# Autodesk Inventor assembly: OpticsTable_Shelf
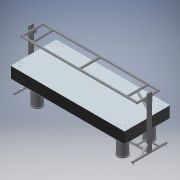
[picture p0: Inventor's stored thumbnail of the model, 180x180]
Saved by Autodesk Inventor 2018 (Build 220112000, 112)
## iProperties
Created: 2018-01-27
Part Number: OpticsTable_Shelf
Document SubType Name: Assembly
Designer: Rich
Author: Rich
## Documents named in this file (23)
- C:\Users\Rich\development\UWaterloo\opticstable_shelf\OpticsTable_Shelf.iam
- C:\Users\Rich\development\UWaterloo\opticstable_shelf\8020-1545-S-1545-S X 54.ipt
- C:\Users\Rich\development\UWaterloo\opticstable_shelf\8020-1515-LS-1515-LS X 24.ipt
- C:\Users\Rich\development\UWaterloo\opticstable_shelf\8020-1515-LS-1515-LS X 21.ipt
- C:\Users\Rich\development\UWaterloo\opticstable_shelf\8020 Original Parts\8020-3660-DEFAULT.ipt
- C:\Users\Rich\development\UWaterloo\opticstable_shelf\8020-1515-LS-1515-LS X 36.ipt
- C:\Users\Rich\development\UWaterloo\opticstable_shelf\8020 Original Parts\8020-2561-$PARTNUMBER.ipt
- C:\Users\Rich\development\UWaterloo\opticstable_shelf\8020 Original Parts\8020-2563-$PARTNUMBER.ipt
- C:\Users\Rich\development\UWaterloo\opticstable_shelf\8020 Original Parts\8020-2190-DEFAULT.ipt
- C:\Users\Rich\development\UWaterloo\opticstable_shelf\8020 Original Parts\8020-2200-DEFAULT.ipt
- C:\Users\Rich\development\UWaterloo\opticstable_shelf\8020 Original Parts\RS2000-410-12.ipt
- C:\Users\Rich\development\UWaterloo\opticstable_shelf\8020 Original Parts\Newport SL 1200-422.ipt
- C:\Users\Rich\development\UWaterloo\opticstable_shelf\8020-1515-LS-1515-LS X 120.ipt
- C:\Users\Rich\development\UWaterloo\opticstable_shelf\8020-1515-LS-1515-LS X 123.ipt
- C:\Users\Rich\development\UWaterloo\opticstable_shelf\8020 Original Parts\8020-3118-DEFAULT.ipt
- C:\Users\Rich\development\UWaterloo\opticstable_shelf\8020 Original Parts\8020-4461-DEFAULT.ipt
- C:\Users\Rich\development\UWaterloo\opticstable_shelf\8020 Original Parts\8020-4336-BLACK-DEFAULT.ipt
- C:\Users\Rich\development\UWaterloo\opticstable_shelf\8020 Original Parts\User Library-ANSI - BHCS - 0.625_5.5.ipt
- C:\Users\Rich\development\UWaterloo\opticstable_shelf\8020 Original Parts\8020-3202-DEFAULT.ipt
- C:\Users\Rich\development\UWaterloo\opticstable_shelf\8020 Original Parts\8020-3065-DEFAULT.ipt
- C:\Users\Rich\development\UWaterloo\opticstable_shelf\8020 Original Parts\8020-2046-DEFAULT.ipt
- C:\Users\Rich\development\UWaterloo\opticstable_shelf\8020 Original Parts\8020-2030-Plain-DEFAULT.ipt
- C:\Users\Rich\development\UWaterloo\opticstable_shelf\8020 Original Parts\8020-3214-DEFAULT.ipt
## Components (107 placed, 22 different names)
1. 8020-1545-S-1545-S X 54:1 — Mate:12, Flush:21, Flush:22, Flush:26, Mate:18, Mate:25, Flush:29, Mate:26, Flush:33, Flush:41, Mate:36, Angle:10, Flush:42, Mate:37, Angle:11, Mate:50, Flush:53, Mate:81, Mate:82, Mate:118, Mate:120, Mate:167, Mate:168, Mate:169
2. 8020-1545-S-1545-S X 54:2 — Mate:2, Flush:4, Flush:18, Flush:20, Flush:21, Mate:15, Mate:16, Mate:21, Flush:27, Mate:23, Flush:34, Flush:39, Mate:34, Angle:8, Flush:40, Mate:35, Angle:9, Mate:49, Flush:52, Mate:79, Mate:80, Mate:125, Mate:126, Mate:170, Mate:171, Mate:172
3. 8020-1515-LS-1515-LS X 24:1 — Flush:61, Mate:60, Flush:62, Mate:61, Flush:63, Flush:64, Mate:129, Mate:179, Flush:93, Flush:94, Mate:180, Flush:95, Flush:96, Tangent:3
4. 8020-1515-LS-1515-LS X 24:2 — Flush:20, Flush:23, Flush:68, Mate:64, Flush:69, Mate:130, Mate:177, Flush:89, Flush:90, Flush:91, Mate:178, Flush:92
5. 8020-1515-LS-1515-LS X 21:1 — Mate:17, Mate:46, Flush:51, Angle:16, Mate:47, Mate:48, Angle:17, Flush:72, Mate:68, Tangent:2, Mate:71
6. 8020-1515-LS-1515-LS X 21:2 — Flush:23, Mate:44, Flush:49, Angle:14, Mate:45, Flush:50, Angle:15, Flush:67, Mate:63
7. 8020-1515-LS-1515-LS X 21:3 — Mate:19, Flush:47, Mate:42, Angle:12, Flush:48, Mate:43, Angle:13, Mate:62, Flush:65, Tangent:1, Mate:67
8. 8020-1515-LS-1515-LS X 36:1 — Mate:12, Flush:19, Flush:22, Mate:24, Mate:27, Flush:30, Mate:38, Flush:43, Mate:39, Flush:44, Flush:77, Mate:75, Mate:175, Flush:85, Flush:86, Mate:176, Flush:87, Flush:88
9. 8020-1515-LS-1515-LS X 36:2 — Mate:1, Mate:2, Flush:4, Flush:18, Flush:19, Mate:20, Mate:22, Flush:28, Mate:40, Flush:45, Mate:41, Flush:46, Mate:72, Flush:75, Mate:173, Flush:81, Flush:82, Mate:174, Flush:83, Flush:84
10. 8020-3660-DEFAULT:1 — Mate:66, Flush:71, Angle:18
11. 8020-3660-DEFAULT:2 — Mate:69, Flush:73, Angle:19
12. 8020-2561-$PARTNUMBER:1 — Mate:22, Mate:23, Flush:28
13. 8020-2561-$PARTNUMBER:2 — Mate:24, Mate:25, Flush:29
14. 8020-2563-$PARTNUMBER:1 — Mate:16, Mate:17, Flush:34, Tangent:1, Mate:67
15. 8020-2563-$PARTNUMBER:2 — Mate:18, Mate:19, Flush:33, Mate:68, Tangent:2
16. 8020-2561-$PARTNUMBER:3 — Mate:26, Mate:27, Flush:30
17. 8020-2561-$PARTNUMBER:4 — Mate:20, Mate:21, Flush:27
18. 8020-2190-DEFAULT:1
19. 8020-2190-DEFAULT:2
20. 8020-2190-DEFAULT:3
21. 8020-3660-DEFAULT:3 — Mate:70, Flush:74, Angle:20
22. 8020-3660-DEFAULT:4 — Mate:65, Flush:70
23. 8020-3660-DEFAULT:9 — Flush:39, Mate:34, Angle:8
24. 8020-3660-DEFAULT:10 — Flush:40, Mate:35, Angle:9
25. 8020-3660-DEFAULT:11 — Flush:41, Mate:36, Angle:10
26. 8020-3660-DEFAULT:12 — Flush:42, Mate:37, Angle:11
27. 8020-2200-DEFAULT:1 — Mate:38, Flush:43
28. 8020-2200-DEFAULT:2 — Mate:39, Flush:44
29. 8020-2200-DEFAULT:3 — Mate:40, Flush:45
30. 8020-2200-DEFAULT:4 — Mate:41, Flush:46
31. 8020-3660-DEFAULT:13 — Flush:47, Mate:42, Angle:12
32. 8020-3660-DEFAULT:14 — Flush:48, Mate:43, Angle:13
33. 8020-3660-DEFAULT:15 — Mate:44, Flush:49, Angle:14
34. 8020-3660-DEFAULT:16 — Mate:45, Flush:50, Angle:15
35. 8020-3660-DEFAULT:17 — Mate:46, Flush:51, Angle:16
36. 8020-3660-DEFAULT:18 — Mate:47, Mate:48, Angle:17
37. 8020-2563-$PARTNUMBER:3 — Mate:49, Flush:52, Flush:76, Mate:73
38. 8020-2563-$PARTNUMBER:4 — Mate:50, Flush:53, Mate:74
39. 8020-2200-DEFAULT:5 — Mate:76, Flush:78
40. 8020-2200-DEFAULT:6 — Flush:79, Mate:77
41. RS2000-410-12:1 — Mate:57, Mate:58, Flush:60
42. 8020-1515-LS-1515-LS X 120:1 — Flush:62, Mate:61, Flush:63, Mate:63, Mate:66, Flush:71, Angle:18, Mate:69, Flush:73, Angle:19, Mate:71
43. 8020-1515-LS-1515-LS X 120:2 — Flush:61, Mate:60, Flush:64, Mate:62, Flush:65, Flush:67, Flush:68, Mate:64, Flush:69, Mate:65, Flush:70, Flush:72, Mate:70, Flush:74, Angle:20
44. 8020-1515-LS-1515-LS X 123:1 — Mate:72, Flush:75, Flush:76, Mate:73, Mate:74, Flush:77, Mate:75, Mate:76, Flush:78, Flush:79, Mate:77, Mate:78, Flush:80
45. 8020-2200-DEFAULT:7 — Mate:78, Flush:80
46. 8020-3118-DEFAULT:1 — Mate:84, Mate:85, Mate:88, Mate:184
47. 8020-4461-DEFAULT:1 — Mate:79, Mate:95, Mate:96, Mate:97, Mate:116, Mate:117, Mate:123, Mate:124, Mate:193, Mate:194
48. 8020-4461-DEFAULT:2 — Mate:80, Mate:83, Mate:88, Mate:89, Mate:127, Mate:128, Mate:195, Mate:196, Mate:198, Mate:200
49. 8020-4461-DEFAULT:3 — Mate:81, Mate:109, Mate:110, Mate:111, Mate:112, Mate:114, Mate:115, Mate:119, Mate:189, Mate:190
50. 8020-4461-DEFAULT:4 — Mate:82, Mate:102, Mate:103, Mate:104, Mate:121, Mate:122, Mate:191, Mate:192, Mate:202, Mate:204
51. 8020-4336-BLACK-DEFAULT:1 — Mate:83, Mate:84, Mate:85, Mate:86, Mate:87, Mate:130, Mate:149, Mate:150, Mate:154, Mate:155, Mate:156
52. 8020-3118-DEFAULT:2 — Mate:86, Mate:87, Mate:89, Mate:185
53. 8020-4336-BLACK-DEFAULT:2 — Mate:91, Mate:92, Mate:93, Mate:94, Mate:95, Mate:151, Mate:152, Mate:153, Mate:157, Mate:158
54. 8020-3118-DEFAULT:3 — Mate:91, Mate:92, Mate:97, Mate:186
55. 8020-3118-DEFAULT:4 — Mate:93, Mate:94, Mate:96, Mate:187
56. 8020-3118-DEFAULT:5 — Mate:98, Mate:99, Mate:104, Mate:181
57. 8020-4336-BLACK-DEFAULT:3 — Mate:98, Mate:99, Mate:100, Mate:101, Mate:102, Mate:129, Mate:159, Mate:160, Mate:161, Mate:162
58. 8020-3118-DEFAULT:6 — Mate:100, Mate:101, Mate:103, Mate:182
59. 8020-4336-BLACK-DEFAULT:4 — Mate:105, Mate:106, Mate:107, Mate:108, Mate:109, Mate:163, Mate:164, Mate:165, Mate:166
60. 8020-3118-DEFAULT:7 — Mate:105, Mate:106, Mate:110, Mate:183
61. 8020-3118-DEFAULT:8 — Mate:107, Mate:108, Mate:111, Mate:188
62. User Library-ANSI - BHCS - 0.625_5.5:1 — Mate:114, Mate:115, Mate:118, Mate:121, Mate:203
63. User Library-ANSI - BHCS - 0.625_5.5:2 — Mate:112, Mate:119, Mate:120, Mate:122, Mate:201
64. User Library-ANSI - BHCS - 0.625_5.5:3 — Mate:117, Mate:124, Mate:125, Mate:128, Mate:199
65. User Library-ANSI - BHCS - 0.625_5.5:4 — Mate:116, Mate:123, Mate:126, Mate:127, Mate:197
66. 8020-3202-DEFAULT:1 — Mate:131, Mate:132
67. 8020-3065-DEFAULT:1 — Mate:131, Mate:132, Mate:159, Mate:160
68. 8020-3202-DEFAULT:2
69. 8020-3065-DEFAULT:2 — Mate:163, Mate:164
70. 8020-3202-DEFAULT:4
71. 8020-3065-DEFAULT:4 — Mate:165, Mate:166
72. 8020-3202-DEFAULT:5
73. 8020-3065-DEFAULT:5 — Mate:161, Mate:162, Tangent:3
74. 8020-3202-DEFAULT:6
75. 8020-3065-DEFAULT:6 — Mate:151, Mate:157, Mate:158
76. 8020-3202-DEFAULT:7
77. 8020-3065-DEFAULT:7 — Mate:150, Mate:155, Mate:156
78. 8020-3202-DEFAULT:8
79. 8020-3065-DEFAULT:8 — Mate:149, Mate:154
80. 8020-3202-DEFAULT:9
81. 8020-3065-DEFAULT:9 — Mate:152, Mate:153
82. 8020-2046-DEFAULT:1 — Mate:167, Mate:168, Mate:169
83. 8020-2046-DEFAULT:2 — Mate:170, Mate:171, Mate:172
84. 8020-2030-Plain-DEFAULT:1 — Mate:180, Flush:95, Flush:96
85. 8020-2030-Plain-DEFAULT:2 — Mate:179, Flush:93, Flush:94
86. 8020-2030-Plain-DEFAULT:3 — Flush:91, Mate:178, Flush:92
87. 8020-2030-Plain-DEFAULT:4 — Mate:177, Flush:89, Flush:90
88. 8020-2030-Plain-DEFAULT:5 — Mate:173, Flush:81, Flush:82
89. 8020-2030-Plain-DEFAULT:6 — Mate:174, Flush:83, Flush:84
90. 8020-2030-Plain-DEFAULT:7 — Mate:175, Flush:85, Flush:86
91. 8020-2030-Plain-DEFAULT:8 — Mate:176, Flush:87, Flush:88
92. 8020-3214-DEFAULT:1 — Mate:181, Mate:191
93. 8020-3214-DEFAULT:2 — Mate:182, Mate:192
94. 8020-3214-DEFAULT:3 — Mate:183, Mate:190
95. 8020-3214-DEFAULT:4 — Mate:185, Mate:196
96. 8020-3214-DEFAULT:5 — Mate:184, Mate:195
97. 8020-3214-DEFAULT:6 — Mate:186, Mate:193
98. 8020-3214-DEFAULT:7 — Mate:187, Mate:194
99. 8020-3214-DEFAULT:8 — Mate:188, Mate:189
100. 8020-3214-DEFAULT:9 — Mate:197, Mate:198
101. 8020-3214-DEFAULT:10 — Mate:199, Mate:200
102. 8020-3214-DEFAULT:11 — Mate:201, Mate:202
103. 8020-3214-DEFAULT:12 — Mate:203, Mate:204
104. Newport SL 1200-422:1 — Mate:57, Mate:58, Flush:60, Mate:59
105. Newport SL 1200-422:2
106. Newport SL 1200-422:3
107. Newport SL 1200-422:4
## Component patterns: (4 elements, first: Newport SL 1200-422:1)
## Relationships (258: Mate 177, Flush 65, Angle 13, Tangent 3)
- Mate:1: 8020-1515-LS-1515-LS X 36:2
- Mate:2: 8020-1545-S-1545-S X 54:2 ↔ 8020-1515-LS-1515-LS X 36:2
- Flush:4: 8020-1545-S-1545-S X 54:2 ↔ 8020-1515-LS-1515-LS X 36:2
- Mate:12: 8020-1545-S-1545-S X 54:1 ↔ 8020-1515-LS-1515-LS X 36:1
- Flush:18 (-400.05 mm): 8020-1545-S-1545-S X 54:2 ↔ 8020-1515-LS-1515-LS X 36:2
- Flush:19: 8020-1515-LS-1515-LS X 36:1 ↔ 8020-1515-LS-1515-LS X 36:2
- Flush:20 (247.65 mm): 8020-1545-S-1545-S X 54:2 ↔ 8020-1515-LS-1515-LS X 24:2
- Flush:21: 8020-1545-S-1545-S X 54:1 ↔ 8020-1545-S-1545-S X 54:2
- Flush:22: 8020-1545-S-1545-S X 54:1 ↔ 8020-1515-LS-1515-LS X 36:1
- Flush:23 (-1530.95 mm): 8020-1515-LS-1515-LS X 24:2 ↔ 8020-1515-LS-1515-LS X 21:2
- Flush:26: 8020-1545-S-1545-S X 54:1
- Mate:15: 8020-1545-S-1545-S X 54:2
- Mate:16: 8020-1545-S-1545-S X 54:2 ↔ 8020-2563-$PARTNUMBER:1
- Mate:17: 8020-1515-LS-1515-LS X 21:1 ↔ 8020-2563-$PARTNUMBER:1
- Mate:18: 8020-1545-S-1545-S X 54:1 ↔ 8020-2563-$PARTNUMBER:2
- Mate:19: 8020-1515-LS-1515-LS X 21:3 ↔ 8020-2563-$PARTNUMBER:2
- Mate:20: 8020-1515-LS-1515-LS X 36:2 ↔ 8020-2561-$PARTNUMBER:4
- Mate:21: 8020-1545-S-1545-S X 54:2 ↔ 8020-2561-$PARTNUMBER:4
- Flush:27: 8020-1545-S-1545-S X 54:2 ↔ 8020-2561-$PARTNUMBER:4
- Mate:22: 8020-1515-LS-1515-LS X 36:2 ↔ 8020-2561-$PARTNUMBER:1
- Mate:23: 8020-1545-S-1545-S X 54:2 ↔ 8020-2561-$PARTNUMBER:1
- Flush:28: 8020-1515-LS-1515-LS X 36:2 ↔ 8020-2561-$PARTNUMBER:1
- Mate:24: 8020-1515-LS-1515-LS X 36:1 ↔ 8020-2561-$PARTNUMBER:2
- Mate:25: 8020-1545-S-1545-S X 54:1 ↔ 8020-2561-$PARTNUMBER:2
- Flush:29: 8020-1545-S-1545-S X 54:1 ↔ 8020-2561-$PARTNUMBER:2
- Mate:26: 8020-1545-S-1545-S X 54:1 ↔ 8020-2561-$PARTNUMBER:3
- Mate:27: 8020-1515-LS-1515-LS X 36:1 ↔ 8020-2561-$PARTNUMBER:3
- Flush:30: 8020-1515-LS-1515-LS X 36:1 ↔ 8020-2561-$PARTNUMBER:3
- Flush:33 (38.1 mm): 8020-1545-S-1545-S X 54:1 ↔ 8020-2563-$PARTNUMBER:2
- Flush:34 (-38.1 mm): 8020-1545-S-1545-S X 54:2 ↔ 8020-2563-$PARTNUMBER:1
- Flush:39: 8020-1545-S-1545-S X 54:2 ↔ 8020-3660-DEFAULT:9
- Mate:34: 8020-1545-S-1545-S X 54:2 ↔ 8020-3660-DEFAULT:9
- Angle:8 (0 deg): 8020-1545-S-1545-S X 54:2 ↔ 8020-3660-DEFAULT:9
- Flush:40: 8020-1545-S-1545-S X 54:2 ↔ 8020-3660-DEFAULT:10
- Mate:35: 8020-1545-S-1545-S X 54:2 ↔ 8020-3660-DEFAULT:10
- Angle:9 (0 deg): 8020-1545-S-1545-S X 54:2 ↔ 8020-3660-DEFAULT:10
- Flush:41: 8020-1545-S-1545-S X 54:1 ↔ 8020-3660-DEFAULT:11
- Mate:36: 8020-1545-S-1545-S X 54:1 ↔ 8020-3660-DEFAULT:11
- Angle:10 (180 deg): 8020-1545-S-1545-S X 54:1 ↔ 8020-3660-DEFAULT:11
- Flush:42: 8020-1545-S-1545-S X 54:1 ↔ 8020-3660-DEFAULT:12
- Mate:37: 8020-1545-S-1545-S X 54:1 ↔ 8020-3660-DEFAULT:12
- Angle:11 (180 deg): 8020-1545-S-1545-S X 54:1 ↔ 8020-3660-DEFAULT:12
- Mate:38: 8020-1515-LS-1515-LS X 36:1 ↔ 8020-2200-DEFAULT:1
- Flush:43 (-38.1 mm): 8020-1515-LS-1515-LS X 36:1 ↔ 8020-2200-DEFAULT:1
- Mate:39: 8020-1515-LS-1515-LS X 36:1 ↔ 8020-2200-DEFAULT:2
- Flush:44 (38.1 mm): 8020-1515-LS-1515-LS X 36:1 ↔ 8020-2200-DEFAULT:2
- Mate:40: 8020-1515-LS-1515-LS X 36:2 ↔ 8020-2200-DEFAULT:3
- Flush:45 (38.1 mm): 8020-1515-LS-1515-LS X 36:2 ↔ 8020-2200-DEFAULT:3
- Mate:41: 8020-1515-LS-1515-LS X 36:2 ↔ 8020-2200-DEFAULT:4
- Flush:46 (38.1 mm): 8020-1515-LS-1515-LS X 36:2 ↔ 8020-2200-DEFAULT:4
- Flush:47: 8020-1515-LS-1515-LS X 21:3 ↔ 8020-3660-DEFAULT:13
- Mate:42: 8020-1515-LS-1515-LS X 21:3 ↔ 8020-3660-DEFAULT:13
- Angle:12 (0 deg): 8020-1515-LS-1515-LS X 21:3 ↔ 8020-3660-DEFAULT:13
- Flush:48: 8020-1515-LS-1515-LS X 21:3 ↔ 8020-3660-DEFAULT:14
- Mate:43: 8020-1515-LS-1515-LS X 21:3 ↔ 8020-3660-DEFAULT:14
- Angle:13 (180 deg): 8020-1515-LS-1515-LS X 21:3 ↔ 8020-3660-DEFAULT:14
- Mate:44: 8020-1515-LS-1515-LS X 21:2 ↔ 8020-3660-DEFAULT:15
- Flush:49: 8020-1515-LS-1515-LS X 21:2 ↔ 8020-3660-DEFAULT:15
- Angle:14 (0 deg): 8020-1515-LS-1515-LS X 21:2 ↔ 8020-3660-DEFAULT:15
- Mate:45: 8020-1515-LS-1515-LS X 21:2 ↔ 8020-3660-DEFAULT:16
- Flush:50: 8020-1515-LS-1515-LS X 21:2 ↔ 8020-3660-DEFAULT:16
- Angle:15 (180 deg): 8020-1515-LS-1515-LS X 21:2 ↔ 8020-3660-DEFAULT:16
- Mate:46: 8020-1515-LS-1515-LS X 21:1 ↔ 8020-3660-DEFAULT:17
- Flush:51: 8020-1515-LS-1515-LS X 21:1 ↔ 8020-3660-DEFAULT:17
- Angle:16 (0 deg): 8020-1515-LS-1515-LS X 21:1 ↔ 8020-3660-DEFAULT:17
- Mate:47: 8020-1515-LS-1515-LS X 21:1 ↔ 8020-3660-DEFAULT:18
- Mate:48: 8020-1515-LS-1515-LS X 21:1 ↔ 8020-3660-DEFAULT:18
- Angle:17 (180 deg): 8020-1515-LS-1515-LS X 21:1 ↔ 8020-3660-DEFAULT:18
- Mate:49: 8020-1545-S-1545-S X 54:2 ↔ 8020-2563-$PARTNUMBER:3
- Flush:52 (38.1 mm): 8020-1545-S-1545-S X 54:2 ↔ 8020-2563-$PARTNUMBER:3
- Mate:50: 8020-1545-S-1545-S X 54:1 ↔ 8020-2563-$PARTNUMBER:4
- Flush:53 (38.1 mm): 8020-1545-S-1545-S X 54:1 ↔ 8020-2563-$PARTNUMBER:4
- Mate:57: RS2000-410-12:1 ↔ Newport SL 1200-422:1
- Mate:58 (-457.2 mm): RS2000-410-12:1 ↔ Newport SL 1200-422:1
- Flush:60 (254 mm): RS2000-410-12:1 ↔ Newport SL 1200-422:1
- Mate:59: Newport SL 1200-422:1
- Flush:61: 8020-1515-LS-1515-LS X 24:1 ↔ 8020-1515-LS-1515-LS X 120:2
- Mate:60: 8020-1515-LS-1515-LS X 24:1 ↔ 8020-1515-LS-1515-LS X 120:2
- Flush:62: 8020-1515-LS-1515-LS X 24:1 ↔ 8020-1515-LS-1515-LS X 120:1
- Mate:61: 8020-1515-LS-1515-LS X 24:1 ↔ 8020-1515-LS-1515-LS X 120:1
- Flush:63: 8020-1515-LS-1515-LS X 24:1 ↔ 8020-1515-LS-1515-LS X 120:1
- Flush:64: 8020-1515-LS-1515-LS X 24:1 ↔ 8020-1515-LS-1515-LS X 120:2
- Mate:62: 8020-1515-LS-1515-LS X 21:3 ↔ 8020-1515-LS-1515-LS X 120:2
- Flush:65: 8020-1515-LS-1515-LS X 21:3 ↔ 8020-1515-LS-1515-LS X 120:2
- Flush:67: 8020-1515-LS-1515-LS X 21:2 ↔ 8020-1515-LS-1515-LS X 120:2
- Mate:63: 8020-1515-LS-1515-LS X 21:2 ↔ 8020-1515-LS-1515-LS X 120:1
- Flush:68: 8020-1515-LS-1515-LS X 24:2 ↔ 8020-1515-LS-1515-LS X 120:2
- Mate:64: 8020-1515-LS-1515-LS X 24:2 ↔ 8020-1515-LS-1515-LS X 120:2
- Flush:69: 8020-1515-LS-1515-LS X 24:2 ↔ 8020-1515-LS-1515-LS X 120:2
- Mate:65: 8020-3660-DEFAULT:4 ↔ 8020-1515-LS-1515-LS X 120:2
- Flush:70: 8020-3660-DEFAULT:4 ↔ 8020-1515-LS-1515-LS X 120:2
- Mate:66: 8020-3660-DEFAULT:1 ↔ 8020-1515-LS-1515-LS X 120:1
- Flush:71: 8020-3660-DEFAULT:1 ↔ 8020-1515-LS-1515-LS X 120:1
- Angle:18 (0 deg): 8020-3660-DEFAULT:1 ↔ 8020-1515-LS-1515-LS X 120:1
- Tangent:1: 8020-1515-LS-1515-LS X 21:3 ↔ 8020-2563-$PARTNUMBER:1
- Mate:67: 8020-1515-LS-1515-LS X 21:3 ↔ 8020-2563-$PARTNUMBER:1
- Flush:72: 8020-1515-LS-1515-LS X 21:1 ↔ 8020-1515-LS-1515-LS X 120:2
- Mate:68: 8020-1515-LS-1515-LS X 21:1 ↔ 8020-2563-$PARTNUMBER:2
- Tangent:2: 8020-1515-LS-1515-LS X 21:1 ↔ 8020-2563-$PARTNUMBER:2
- Mate:69: 8020-3660-DEFAULT:2 ↔ 8020-1515-LS-1515-LS X 120:1
- Flush:73: 8020-3660-DEFAULT:2 ↔ 8020-1515-LS-1515-LS X 120:1
- Angle:19 (180 deg): 8020-3660-DEFAULT:2 ↔ 8020-1515-LS-1515-LS X 120:1
- Mate:70: 8020-3660-DEFAULT:3 ↔ 8020-1515-LS-1515-LS X 120:2
- Flush:74: 8020-3660-DEFAULT:3 ↔ 8020-1515-LS-1515-LS X 120:2
- Angle:20 (0 deg): 8020-3660-DEFAULT:3 ↔ 8020-1515-LS-1515-LS X 120:2
- Mate:71: 8020-1515-LS-1515-LS X 21:1 ↔ 8020-1515-LS-1515-LS X 120:1
- Mate:72: 8020-1515-LS-1515-LS X 36:2 ↔ 8020-1515-LS-1515-LS X 123:1
- Flush:75: 8020-1515-LS-1515-LS X 36:2 ↔ 8020-1515-LS-1515-LS X 123:1
- Flush:76: 8020-2563-$PARTNUMBER:3 ↔ 8020-1515-LS-1515-LS X 123:1
- Mate:73: 8020-2563-$PARTNUMBER:3 ↔ 8020-1515-LS-1515-LS X 123:1
- Mate:74: 8020-2563-$PARTNUMBER:4 ↔ 8020-1515-LS-1515-LS X 123:1
- Flush:77: 8020-1515-LS-1515-LS X 36:1 ↔ 8020-1515-LS-1515-LS X 123:1
- Mate:75: 8020-1515-LS-1515-LS X 36:1 ↔ 8020-1515-LS-1515-LS X 123:1
- Mate:76: 8020-2200-DEFAULT:5 ↔ 8020-1515-LS-1515-LS X 123:1
- Flush:78 (38.1 mm): 8020-2200-DEFAULT:5 ↔ 8020-1515-LS-1515-LS X 123:1
- Flush:79 (-38.1 mm): 8020-2200-DEFAULT:6 ↔ 8020-1515-LS-1515-LS X 123:1
- Mate:77: 8020-2200-DEFAULT:6 ↔ 8020-1515-LS-1515-LS X 123:1
- Mate:78: 8020-1515-LS-1515-LS X 123:1 ↔ 8020-2200-DEFAULT:7
- Flush:80 (38.1 mm): 8020-1515-LS-1515-LS X 123:1 ↔ 8020-2200-DEFAULT:7
- Mate:79: 8020-1545-S-1545-S X 54:2 ↔ 8020-4461-DEFAULT:1
- Mate:80: 8020-1545-S-1545-S X 54:2 ↔ 8020-4461-DEFAULT:2
- Mate:81: 8020-1545-S-1545-S X 54:1 ↔ 8020-4461-DEFAULT:3
- Mate:82: 8020-1545-S-1545-S X 54:1 ↔ 8020-4461-DEFAULT:4
- Mate:83: 8020-4461-DEFAULT:2 ↔ 8020-4336-BLACK-DEFAULT:1
- Mate:84: 8020-3118-DEFAULT:1 ↔ 8020-4336-BLACK-DEFAULT:1
- Mate:85: 8020-3118-DEFAULT:1 ↔ 8020-4336-BLACK-DEFAULT:1
- Mate:86: 8020-4336-BLACK-DEFAULT:1 ↔ 8020-3118-DEFAULT:2
- Mate:87: 8020-4336-BLACK-DEFAULT:1 ↔ 8020-3118-DEFAULT:2
- Mate:88: 8020-3118-DEFAULT:1 ↔ 8020-4461-DEFAULT:2
- Mate:89: 8020-4461-DEFAULT:2 ↔ 8020-3118-DEFAULT:2
- Mate:91: 8020-4336-BLACK-DEFAULT:2 ↔ 8020-3118-DEFAULT:3
- Mate:92: 8020-4336-BLACK-DEFAULT:2 ↔ 8020-3118-DEFAULT:3
- Mate:93: 8020-4336-BLACK-DEFAULT:2 ↔ 8020-3118-DEFAULT:4
- Mate:94: 8020-4336-BLACK-DEFAULT:2 ↔ 8020-3118-DEFAULT:4
- Mate:95: 8020-4461-DEFAULT:1 ↔ 8020-4336-BLACK-DEFAULT:2
- Mate:96: 8020-4461-DEFAULT:1 ↔ 8020-3118-DEFAULT:4
- Mate:97: 8020-4461-DEFAULT:1 ↔ 8020-3118-DEFAULT:3
- Mate:98: 8020-3118-DEFAULT:5 ↔ 8020-4336-BLACK-DEFAULT:3
- Mate:99: 8020-3118-DEFAULT:5 ↔ 8020-4336-BLACK-DEFAULT:3
- Mate:100: 8020-4336-BLACK-DEFAULT:3 ↔ 8020-3118-DEFAULT:6
- Mate:101: 8020-4336-BLACK-DEFAULT:3 ↔ 8020-3118-DEFAULT:6
- Mate:102: 8020-4461-DEFAULT:4 ↔ 8020-4336-BLACK-DEFAULT:3
- Mate:103: 8020-4461-DEFAULT:4 ↔ 8020-3118-DEFAULT:6
- Mate:104: 8020-4461-DEFAULT:4 ↔ 8020-3118-DEFAULT:5
- Mate:105: 8020-4336-BLACK-DEFAULT:4 ↔ 8020-3118-DEFAULT:7
- Mate:106: 8020-4336-BLACK-DEFAULT:4 ↔ 8020-3118-DEFAULT:7
- Mate:107: 8020-4336-BLACK-DEFAULT:4 ↔ 8020-3118-DEFAULT:8
- Mate:108: 8020-4336-BLACK-DEFAULT:4 ↔ 8020-3118-DEFAULT:8
- Mate:109: 8020-4461-DEFAULT:3 ↔ 8020-4336-BLACK-DEFAULT:4
- Mate:110: 8020-4461-DEFAULT:3 ↔ 8020-3118-DEFAULT:7
- Mate:111: 8020-4461-DEFAULT:3 ↔ 8020-3118-DEFAULT:8
- Mate:112: 8020-4461-DEFAULT:3 ↔ User Library-ANSI - BHCS - 0.625_5.5:2
- Mate:114: 8020-4461-DEFAULT:3 ↔ User Library-ANSI - BHCS - 0.625_5.5:1
- Mate:115: 8020-4461-DEFAULT:3 ↔ User Library-ANSI - BHCS - 0.625_5.5:1
- Mate:116: 8020-4461-DEFAULT:1 ↔ User Library-ANSI - BHCS - 0.625_5.5:4
- Mate:117: 8020-4461-DEFAULT:1 ↔ User Library-ANSI - BHCS - 0.625_5.5:3
- Mate:118: 8020-1545-S-1545-S X 54:1 ↔ User Library-ANSI - BHCS - 0.625_5.5:1
- Mate:119: 8020-4461-DEFAULT:3 ↔ User Library-ANSI - BHCS - 0.625_5.5:2
- Mate:120: 8020-1545-S-1545-S X 54:1 ↔ User Library-ANSI - BHCS - 0.625_5.5:2
- Mate:121: 8020-4461-DEFAULT:4 ↔ User Library-ANSI - BHCS - 0.625_5.5:1
- Mate:122: 8020-4461-DEFAULT:4 ↔ User Library-ANSI - BHCS - 0.625_5.5:2
- Mate:123: 8020-4461-DEFAULT:1 ↔ User Library-ANSI - BHCS - 0.625_5.5:4
- Mate:124: 8020-4461-DEFAULT:1 ↔ User Library-ANSI - BHCS - 0.625_5.5:3
- Mate:125: 8020-1545-S-1545-S X 54:2 ↔ User Library-ANSI - BHCS - 0.625_5.5:3
- Mate:126: 8020-1545-S-1545-S X 54:2 ↔ User Library-ANSI - BHCS - 0.625_5.5:4
- Mate:127: 8020-4461-DEFAULT:2 ↔ User Library-ANSI - BHCS - 0.625_5.5:4
- Mate:128: 8020-4461-DEFAULT:2 ↔ User Library-ANSI - BHCS - 0.625_5.5:3
- Mate:129: 8020-1515-LS-1515-LS X 24:1 ↔ 8020-4336-BLACK-DEFAULT:3
- Mate:130: 8020-1515-LS-1515-LS X 24:2 ↔ 8020-4336-BLACK-DEFAULT:1
- Mate:131: 8020-3202-DEFAULT:1 ↔ 8020-3065-DEFAULT:1
- Mate:132 (12.7 mm): 8020-3202-DEFAULT:1 ↔ 8020-3065-DEFAULT:1
- [Mate]: 8020-3202-DEFAULT:2 ↔ 8020-3065-DEFAULT:2
- [Mate] (12.7 mm): 8020-3202-DEFAULT:2 ↔ 8020-3065-DEFAULT:2
- [Mate]: 8020-3202-DEFAULT:4 ↔ 8020-3065-DEFAULT:4
- [Mate] (12.7 mm): 8020-3202-DEFAULT:4 ↔ 8020-3065-DEFAULT:4
- [Mate]: 8020-3202-DEFAULT:5 ↔ 8020-3065-DEFAULT:5
- [Mate] (12.7 mm): 8020-3202-DEFAULT:5 ↔ 8020-3065-DEFAULT:5
- [Mate]: 8020-3202-DEFAULT:6 ↔ 8020-3065-DEFAULT:6
- [Mate] (12.7 mm): 8020-3202-DEFAULT:6 ↔ 8020-3065-DEFAULT:6
- [Mate]: 8020-3202-DEFAULT:7 ↔ 8020-3065-DEFAULT:7
- [Mate] (12.7 mm): 8020-3202-DEFAULT:7 ↔ 8020-3065-DEFAULT:7
- [Mate]: 8020-3202-DEFAULT:8 ↔ 8020-3065-DEFAULT:8
- [Mate] (12.7 mm): 8020-3202-DEFAULT:8 ↔ 8020-3065-DEFAULT:8
- [Mate]: 8020-3202-DEFAULT:9 ↔ 8020-3065-DEFAULT:9
- [Mate] (12.7 mm): 8020-3202-DEFAULT:9 ↔ 8020-3065-DEFAULT:9
- Mate:149: 8020-4336-BLACK-DEFAULT:1 ↔ 8020-3065-DEFAULT:8
- Mate:150: 8020-4336-BLACK-DEFAULT:1 ↔ 8020-3065-DEFAULT:7
- Mate:151: 8020-4336-BLACK-DEFAULT:2 ↔ 8020-3065-DEFAULT:6
- Mate:152: 8020-4336-BLACK-DEFAULT:2 ↔ 8020-3065-DEFAULT:9
- Mate:153: 8020-4336-BLACK-DEFAULT:2 ↔ 8020-3065-DEFAULT:9
- Mate:154: 8020-4336-BLACK-DEFAULT:1 ↔ 8020-3065-DEFAULT:8
- Mate:155: 8020-4336-BLACK-DEFAULT:1 ↔ 8020-3065-DEFAULT:7
- Mate:156: 8020-4336-BLACK-DEFAULT:1 ↔ 8020-3065-DEFAULT:7
- Mate:157: 8020-4336-BLACK-DEFAULT:2 ↔ 8020-3065-DEFAULT:6
- Mate:158: 8020-4336-BLACK-DEFAULT:2 ↔ 8020-3065-DEFAULT:6
- Mate:159: 8020-4336-BLACK-DEFAULT:3 ↔ 8020-3065-DEFAULT:1
- Mate:160: 8020-4336-BLACK-DEFAULT:3 ↔ 8020-3065-DEFAULT:1
- Mate:161: 8020-4336-BLACK-DEFAULT:3 ↔ 8020-3065-DEFAULT:5
- Mate:162: 8020-4336-BLACK-DEFAULT:3 ↔ 8020-3065-DEFAULT:5
- Mate:163: 8020-4336-BLACK-DEFAULT:4 ↔ 8020-3065-DEFAULT:2
- Mate:164: 8020-4336-BLACK-DEFAULT:4 ↔ 8020-3065-DEFAULT:2
- Mate:165: 8020-4336-BLACK-DEFAULT:4 ↔ 8020-3065-DEFAULT:4
- Mate:166: 8020-4336-BLACK-DEFAULT:4 ↔ 8020-3065-DEFAULT:4
- Mate:167: 8020-1545-S-1545-S X 54:1 ↔ 8020-2046-DEFAULT:1
- Mate:168: 8020-1545-S-1545-S X 54:1 ↔ 8020-2046-DEFAULT:1
- Mate:169: 8020-1545-S-1545-S X 54:1 ↔ 8020-2046-DEFAULT:1
- Mate:170: 8020-1545-S-1545-S X 54:2 ↔ 8020-2046-DEFAULT:2
- Mate:171: 8020-1545-S-1545-S X 54:2 ↔ 8020-2046-DEFAULT:2
- Mate:172: 8020-1545-S-1545-S X 54:2 ↔ 8020-2046-DEFAULT:2
- Mate:173: 8020-1515-LS-1515-LS X 36:2 ↔ 8020-2030-Plain-DEFAULT:5
- Flush:81: 8020-1515-LS-1515-LS X 36:2 ↔ 8020-2030-Plain-DEFAULT:5
- Flush:82: 8020-1515-LS-1515-LS X 36:2 ↔ 8020-2030-Plain-DEFAULT:5
- Mate:174: 8020-1515-LS-1515-LS X 36:2 ↔ 8020-2030-Plain-DEFAULT:6
- Flush:83: 8020-1515-LS-1515-LS X 36:2 ↔ 8020-2030-Plain-DEFAULT:6
- Flush:84: 8020-1515-LS-1515-LS X 36:2 ↔ 8020-2030-Plain-DEFAULT:6
- Mate:175: 8020-1515-LS-1515-LS X 36:1 ↔ 8020-2030-Plain-DEFAULT:7
- Flush:85: 8020-1515-LS-1515-LS X 36:1 ↔ 8020-2030-Plain-DEFAULT:7
- Flush:86: 8020-1515-LS-1515-LS X 36:1 ↔ 8020-2030-Plain-DEFAULT:7
- Mate:176: 8020-1515-LS-1515-LS X 36:1 ↔ 8020-2030-Plain-DEFAULT:8
- Flush:87: 8020-1515-LS-1515-LS X 36:1 ↔ 8020-2030-Plain-DEFAULT:8
- Flush:88: 8020-1515-LS-1515-LS X 36:1 ↔ 8020-2030-Plain-DEFAULT:8
- Mate:177: 8020-1515-LS-1515-LS X 24:2 ↔ 8020-2030-Plain-DEFAULT:4
- Flush:89: 8020-1515-LS-1515-LS X 24:2 ↔ 8020-2030-Plain-DEFAULT:4
- Flush:90: 8020-1515-LS-1515-LS X 24:2 ↔ 8020-2030-Plain-DEFAULT:4
- Flush:91: 8020-1515-LS-1515-LS X 24:2 ↔ 8020-2030-Plain-DEFAULT:3
- Mate:178: 8020-1515-LS-1515-LS X 24:2 ↔ 8020-2030-Plain-DEFAULT:3
- Flush:92: 8020-1515-LS-1515-LS X 24:2 ↔ 8020-2030-Plain-DEFAULT:3
- Mate:179: 8020-1515-LS-1515-LS X 24:1 ↔ 8020-2030-Plain-DEFAULT:2
- Flush:93: 8020-1515-LS-1515-LS X 24:1 ↔ 8020-2030-Plain-DEFAULT:2
- Flush:94: 8020-1515-LS-1515-LS X 24:1 ↔ 8020-2030-Plain-DEFAULT:2
- Mate:180: 8020-1515-LS-1515-LS X 24:1 ↔ 8020-2030-Plain-DEFAULT:1
- Flush:95: 8020-1515-LS-1515-LS X 24:1 ↔ 8020-2030-Plain-DEFAULT:1
- Flush:96: 8020-1515-LS-1515-LS X 24:1 ↔ 8020-2030-Plain-DEFAULT:1
- Tangent:3: 8020-1515-LS-1515-LS X 24:1 ↔ 8020-3065-DEFAULT:5
- Mate:181: 8020-3118-DEFAULT:5 ↔ 8020-3214-DEFAULT:1
- Mate:182: 8020-3118-DEFAULT:6 ↔ 8020-3214-DEFAULT:2
- Mate:183: 8020-3118-DEFAULT:7 ↔ 8020-3214-DEFAULT:3
- Mate:184: 8020-3118-DEFAULT:1 ↔ 8020-3214-DEFAULT:5
- Mate:185: 8020-3118-DEFAULT:2 ↔ 8020-3214-DEFAULT:4
- Mate:186: 8020-3118-DEFAULT:3 ↔ 8020-3214-DEFAULT:6
- Mate:187: 8020-3118-DEFAULT:4 ↔ 8020-3214-DEFAULT:7
- Mate:188: 8020-3118-DEFAULT:8 ↔ 8020-3214-DEFAULT:8
- Mate:189: 8020-4461-DEFAULT:3 ↔ 8020-3214-DEFAULT:8
- Mate:190: 8020-4461-DEFAULT:3 ↔ 8020-3214-DEFAULT:3
- Mate:191: 8020-4461-DEFAULT:4 ↔ 8020-3214-DEFAULT:1
- Mate:192: 8020-4461-DEFAULT:4 ↔ 8020-3214-DEFAULT:2
- Mate:193: 8020-4461-DEFAULT:1 ↔ 8020-3214-DEFAULT:6
- Mate:194: 8020-4461-DEFAULT:1 ↔ 8020-3214-DEFAULT:7
- Mate:195: 8020-4461-DEFAULT:2 ↔ 8020-3214-DEFAULT:5
- Mate:196: 8020-4461-DEFAULT:2 ↔ 8020-3214-DEFAULT:4
- Mate:197: User Library-ANSI - BHCS - 0.625_5.5:4 ↔ 8020-3214-DEFAULT:9
- Mate:198: 8020-4461-DEFAULT:2 ↔ 8020-3214-DEFAULT:9
- Mate:199: User Library-ANSI - BHCS - 0.625_5.5:3 ↔ 8020-3214-DEFAULT:10
- Mate:200: 8020-4461-DEFAULT:2 ↔ 8020-3214-DEFAULT:10
- Mate:201: User Library-ANSI - BHCS - 0.625_5.5:2 ↔ 8020-3214-DEFAULT:11
- Mate:202: 8020-4461-DEFAULT:4 ↔ 8020-3214-DEFAULT:11
- Mate:203: User Library-ANSI - BHCS - 0.625_5.5:1 ↔ 8020-3214-DEFAULT:12
- Mate:204: 8020-4461-DEFAULT:4 ↔ 8020-3214-DEFAULT:12
## Named parameters: d285_d283 = 0 mm, d286_d284 = 12.7 mm, d289_d285_d283 = 0 mm, d290_d286_d284 = 12.7 mm, d291_d285_d283 = 0 mm, d292_d286_d284 = 12.7 mm, d293_d285_d283 = 0 mm, d294_d286_d284 = 12.7 mm, d295_d285_d283 = 0 mm, d296_d286_d284 = 12.7 mm, d297_d285_d283 = 0 mm, d298_d286_d284 = 12.7 mm, d299_d285_d283 = 0 mm, d300_d286_d284 = 12.7 mm
